# Autodesk Inventor assembly: DigitalClockiam
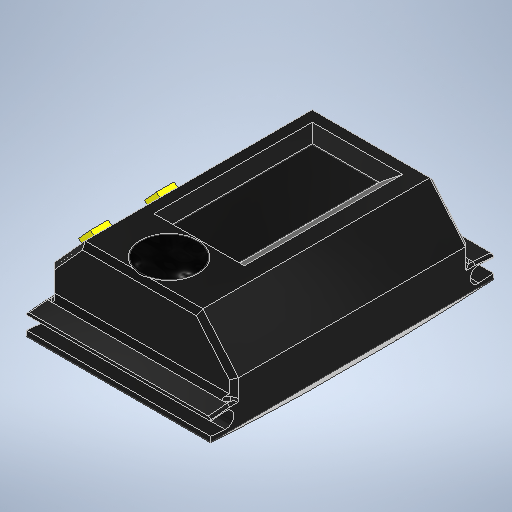
[picture p0: Inventor's stored thumbnail of the model, 512x512]
Saved by Autodesk Inventor 2025.2 (Build 292293000, 293)
## iProperties
Created: 2026-02-19
Part Number: DigitalClockiam
Document SubType Name: Assembly
Designer: naka6
Author: naka6
## iProperties of the stored document OMRON B3F 12mm TACT SWITCH.ipt
Created: 2021-10-02
Part Number: OMRON B3F 12mm TACT SWITCH
Material: 一般
Description: STEP AP214
Document SubType Name: Modeling
Designer: naka6
Density: 1 g/cm^3
Appearance: 既定
Sending System: SolidWorks 2020
Preprocessor: SwSTEP 2.0
Title: OMRON B3F 12mm TACT SWITCH.STEP
Author: Alexrolex
Revision Number: ANY
## iProperties of the stored document ESP32-S3_Zero.ipt
Created: 2025-06-08
Part Number: ESP32-S3_Zero
Material: Steel
Description: STEP AP214
Document SubType Name: Modeling
Designer: naka6
Density: 7.85 g/cm^3
Appearance: 既定
Sending System: Autodesk Translation Framework v14.10.0.0
Preprocessor: ST-DEVELOPER v20.1
Title: ESP32-S3_Zero.step
## iProperties of the stored document Boost 5V 8V 9V 12V_P.ipt
Created: 2025-11-24
Part Number: Boost 5V 8V 9V 12V_P
Material: 一般
Document SubType Name: Modeling
Designer: naka6
Density: 1 g/cm^3
Appearance: 既定
Sending System: SolidWorks 2013
Last Author: Admin
Last Saved: 2025-11-24
Author: naka6
## Documents named in this file (11)
- C:\Users\naka6\Projects\TimeFaker\DigitalClockiam.iam
- C:\Users\naka6\Projects\TimeFaker\HW-069.ipt
- C:\Users\naka6\Projects\TimeFaker\Buzzer.ipt
- **C:\Users\naka6\Projects\TimeFaker\DigitalClockiam.iam*LocalDocs*xAaaaqydaAaaaaaaaAaaaq33sLh*Boost 5V 8V 9V 12V_P.ipt
- **C:\Users\naka6\Projects\TimeFaker\DigitalClockiam.iam*LocalDocs*xAaaaqncaAaaaaaaaAaaaaigj2e*OMRON B3F 12mm TACT SWITCH.ipt
- **C:\Users\naka6\Projects\TimeFaker\DigitalClockiam.iam*LocalDocs*xAaaaamcaAaaaaaaaAaaaaez4Rh*ESP32-S3_Zero.ipt
- C:\Users\naka6\Projects\TimeFaker\batery.ipt
- C:\Users\naka6\Projects\TimeFaker\CaseTop.ipt
- C:\Users\naka6\Projects\TimeFaker\Motor.ipt
- C:\Users\naka6\Projects\TimeFaker\CaseButtom.ipt
- C:\Users\naka6\Projects\TimeFaker\boost-5v-8v-9v-12v-1.snapshot.3\Boost 5V 8V 9V 12V_P.SLDPRT
## Components (10 placed, 9 different names)
1. HW-069:1 — メイト:1, 正接:1, 正接:2, メイト:2, フラッシュ:1, フラッシュ:2, メイト:3, メイト:4, メイト:5, フラッシュ:3, 角度:2, メイト:6, メイト:7, 角度:4, メイト:8
2. Buzzer:1 — メイト:1, 正接:1, 正接:2
3. Boost 5V 8V 9V 12V_P:1 — メイト:3, 角度:1, メイト:4, メイト:5, フラッシュ:3, 角度:3
4. batery:1 — メイト:2, フラッシュ:1, フラッシュ:2, 角度:1, フラッシュ:6, フラッシュ:7, フラッシュ:8
5. OMRON B3F 12mm TACT SWITCH:1 — 角度:2, メイト:6, 角度:3, フラッシュ:4, フラッシュ:5
6. OMRON B3F 12mm TACT SWITCH:2 — メイト:7, 角度:4, フラッシュ:4, フラッシュ:5
7. ESP32-S3_Zero:1 — メイト:8, フラッシュ:6
8. CaseTop:1 — フラッシュ:7, メイト:9
9. Motor:1 — メイト:9
10. CaseButtom:1 — フラッシュ:8
## Relationships (23: Mate 9, Flush 8, Angle 4, Tangent 2)
- メイト:1 [Mate]: HW-069:1 ↔ Buzzer:1
- 正接:1 [Tangent]: HW-069:1 ↔ Buzzer:1
- 正接:2 [Tangent]: HW-069:1 ↔ Buzzer:1
- メイト:2 [Mate] (1.5 mm): HW-069:1 ↔ batery:1
- フラッシュ:1 [Flush]: HW-069:1 ↔ batery:1
- フラッシュ:2 [Flush]: HW-069:1 ↔ batery:1
- メイト:3 [Mate]: HW-069:1 ↔ Boost 5V 8V 9V 12V_P:1
- 角度:1 [Angle] (0 deg): Boost 5V 8V 9V 12V_P:1 ↔ batery:1
- メイト:4 [Mate]: HW-069:1 ↔ Boost 5V 8V 9V 12V_P:1
- メイト:5 [Mate]: HW-069:1 ↔ Boost 5V 8V 9V 12V_P:1
- フラッシュ:3 [Flush]: HW-069:1 ↔ Boost 5V 8V 9V 12V_P:1
- 角度:2 [Angle] (90 deg): HW-069:1 ↔ OMRON B3F 12mm TACT SWITCH:1
- メイト:6 [Mate]: HW-069:1 ↔ OMRON B3F 12mm TACT SWITCH:1
- 角度:3 [Angle] (0 deg): Boost 5V 8V 9V 12V_P:1 ↔ OMRON B3F 12mm TACT SWITCH:1
- メイト:7 [Mate]: HW-069:1 ↔ OMRON B3F 12mm TACT SWITCH:2
- 角度:4 [Angle] (90 deg): HW-069:1 ↔ OMRON B3F 12mm TACT SWITCH:2
- フラッシュ:4 [Flush]: OMRON B3F 12mm TACT SWITCH:1 ↔ OMRON B3F 12mm TACT SWITCH:2
- フラッシュ:5 [Flush]: OMRON B3F 12mm TACT SWITCH:1 ↔ OMRON B3F 12mm TACT SWITCH:2
- メイト:8 [Mate]: HW-069:1 ↔ ESP32-S3_Zero:1
- フラッシュ:6 [Flush]: batery:1 ↔ ESP32-S3_Zero:1
- フラッシュ:7 [Flush]: batery:1 ↔ CaseTop:1
- メイト:9 [Mate]: CaseTop:1 ↔ Motor:1
- フラッシュ:8 [Flush]: batery:1 ↔ CaseButtom:1
